# Autodesk Inventor assembly: Miras
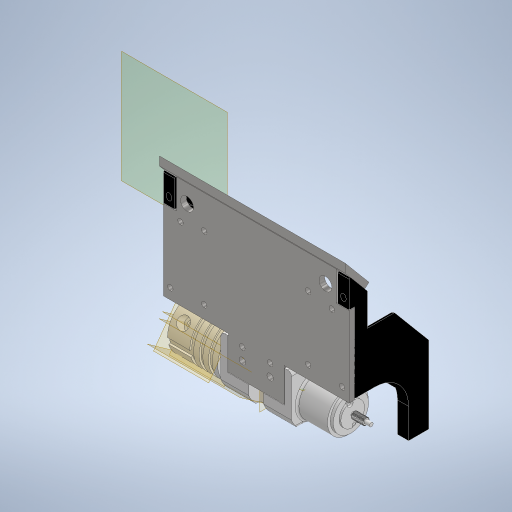
[picture p0: Inventor's stored thumbnail of the model, 512x512]
Saved by Autodesk Inventor 2023.5 (Build 275446000, 446)
## iProperties
Created: 2022-12-28
Part Number: Miras
Document SubType Name: Assembly
Designer: Kamil
Author: Kamil
## Documents named in this file (24)
- E:\PROJECTS_REPOS\Miras\mechanics\Miras.iam
- E:\PROJECTS_REPOS\Miras\mechanics\blacha_stal_3mm.ipt
- E:\PROJECTS_REPOS\Miras\mechanics\steel_2.ipt
- E:\PROJECTS_REPOS\Miras\mechanics\lead_3.ipt
- E:\PROJECTS_REPOS\Miras\mechanics\Part8.ipt
- E:\PROJECTS_REPOS\Miras\mechanics\n20 motor.ipt
- E:\PROJECTS_REPOS\Miras\mechanics\felga.ipt
- E:\PROJECTS_REPOS\Miras\mechanics\opona.ipt
- E:\PROJECTS_REPOS\Miras\mechanics\strug.ipt
- E:\PROJECTS_REPOS\Miras\mechanics\sciana.ipt
- E:\PROJECTS_REPOS\Miras\mechanics\sciana_MIR.ipt
- E:\PROJECTS_REPOS\Miras\mechanics\mirror.ipt
- E:\PROJECTS_REPOS\Miras\mechanics\uchwyt na plytke.ipt
- E:\PROJECTS_REPOS\Miras\mechanics\wachlarz_1.ipt
- E:\PROJECTS_REPOS\Miras\mechanics\montaz_wachlarzy_2.ipt
- E:\PROJECTS_REPOS\Miras\mechanics\wachlarz_1_MIR.ipt
- E:\PROJECTS_REPOS\Miras\mechanics\Serwo_z_widelcem.iam
- E:\PROJECTS_REPOS\Miras\mechanics\widelec.ipt
- E:\PROJECTS_REPOS\Miras\mechanics\faulhaber_motor.ipt
- E:\PROJECTS_REPOS\Miras\mechanics\PCB.ipt
- E:\PROJECTS_REPOS\Miras\mechanics\motors_mount_miras.ipt
- E:\PROJECTS_REPOS\Miras\mechanics\wymiar.ipt
- E:\PROJECTS_REPOS\EX_ONE_minisumo\mechanics\inventor_parts\kolo_tetsowe.ipt
- E:\PROJECTS_REPOS\Miras\mechanics\pcb_podstawka.ipt
## Components (28 placed, 23 different names)
1. blacha_stal_3mm:1 — Mate:1, Mate:2, Mate:27, Flush:4, Flush:5, Mate:28, Flush:6, Mate:30, Flush:7, Flush:22, Zestawiające:65, Kątowe:2, Równoległe:24, Równoległe:25, Równoległe:27, Równoległe:28, Zestawiające:70, Zestawiające:74, Zestawiające:75, Zestawiające:76
2. steel_2:1 — Mate:1, Mate:2, Mate:4, Mate:5, Flush:1, Zestawiające:66
3. lead_3:1 — Mate:4, Mate:5, Flush:1, Flush:2, Flush:3, Mate:16
4. Part8:1 — Flush:2, Flush:3, Mate:11, Mate:12, Mate:13, Mate:14, Mate:15, Mate:18, Mate:37, Flush:9, Flush:10, Mate:55
5. n20 motor:1 — Mate:10, Mate:11, Mate:13, Mate:14, Mate:19, Mate:20, Mate:21
6. n20 motor:2 — Mate:10, Mate:12, Mate:15, Mate:16, Mate:17, Mate:22
7. felga:1 — Mate:17, Mate:18, Mate:22, Mate:24, Mate:25
8. felga:2 — Mate:19, Mate:20, Mate:21, Mate:23, Mate:26
9. opona:1 — Mate:23, Mate:26, Zestawiające:63
10. opona:2 — Mate:24, Mate:25
11. strug:1 — Mate:27, Flush:4, Flush:5, Mate:29, Mate:31, Mate:35, Flush:21, Flush:22, Zestawiające:68, Równoległe:26
12. sciana:1 — Mate:28, Mate:29, Flush:6
13. sciana_MIR:1 — Mate:30, Flush:7, Mate:31, Flush:8, Mate:36
14. mirror:1 — Mate:35, Flush:8, Mate:36, Flush:21
15. uchwyt na plytke:1 — Mate:37, Flush:9, Flush:10, Flush:15, Mate:50, Mate:51, Mate:58
16. montaz_wachlarzy_2:1 — Flush:15, Mate:50, Mate:51, Mate:52, Mate:53, Mate:54
17. wachlarz_1:2 — Mate:52, Mate:53, Flush:16
18. wachlarz_1_MIR:1 — Mate:54, Flush:16
19. widelec:1 — Mate:55, Mate:56, Mate:57
20. Serwo_z_widelcem:1 [sub-assembly] — Mate:56, Mate:57, Mate:58
21. faulhaber_motor:1 — Kątowe:1, Zestawiające:62, Zestawiające:72
22. faulhaber_motor:2 — Kątowe:1, Zestawiające:62, Zestawiające:63, Zestawiające:71, Zestawiające:73
23. PCB:1 — Zestawiające:65, Kątowe:2, Równoległe:24, Zestawiające:66
24. motors_mount_miras:1 — Zestawiające:69, Zestawiające:70, Zestawiające:71, Zestawiające:72, Zestawiające:73
25. wymiar:1 — Zestawiające:68, Równoległe:25, Równoległe:26, Zestawiające:69
26. kolo_tetsowe:1 — Równoległe:27
27. kolo_tetsowe:2 — Równoległe:28
28. pcb_podstawka:1 — Zestawiające:74, Zestawiające:75, Zestawiające:76
## Relationships (72: Mate 51, Flush 19, Angle 2)
- Mate:1: blacha_stal_3mm:1 ↔ steel_2:1
- Mate:2: blacha_stal_3mm:1 ↔ steel_2:1
- Mate:4: steel_2:1 ↔ lead_3:1
- Mate:5: steel_2:1 ↔ lead_3:1
- Flush:1: steel_2:1 ↔ lead_3:1
- Flush:2: lead_3:1 ↔ Part8:1
- Flush:3: lead_3:1 ↔ Part8:1
- Mate:10 (5 mm): n20 motor:1 ↔ n20 motor:2
- Mate:11 (2.5 mm): Part8:1 ↔ n20 motor:1
- Mate:12: Part8:1 ↔ n20 motor:2
- Mate:13: Part8:1 ↔ n20 motor:1
- Mate:14: Part8:1 ↔ n20 motor:1
- Mate:15: Part8:1 ↔ n20 motor:2
- Mate:16: lead_3:1 ↔ n20 motor:2
- Mate:17 (0.5 mm): n20 motor:2 ↔ felga:1
- Mate:18: Part8:1 ↔ felga:1
- Mate:19 (0.5 mm): n20 motor:1 ↔ felga:2
- Mate:20: n20 motor:1 ↔ felga:2
- Mate:21: n20 motor:1 ↔ felga:2
- Mate:22: n20 motor:2 ↔ felga:1
- Mate:23: felga:2 ↔ opona:1
- Mate:24: felga:1 ↔ opona:2
- Mate:25: felga:1 ↔ opona:2
- Mate:26: felga:2 ↔ opona:1
- Mate:27: blacha_stal_3mm:1 ↔ strug:1
- Flush:4: blacha_stal_3mm:1 ↔ strug:1
- Flush:5 (2.1 mm): blacha_stal_3mm:1 ↔ strug:1
- Mate:28: blacha_stal_3mm:1 ↔ sciana:1
- Mate:29: strug:1 ↔ sciana:1
- Flush:6: blacha_stal_3mm:1 ↔ sciana:1
- Mate:30: blacha_stal_3mm:1 ↔ sciana_MIR:1
- Flush:7: blacha_stal_3mm:1 ↔ sciana_MIR:1
- Mate:31: strug:1 ↔ sciana_MIR:1
- Mate:35: strug:1 ↔ mirror:1
- Flush:8: sciana_MIR:1 ↔ mirror:1
- Mate:36: sciana_MIR:1 ↔ mirror:1
- Mate:37: Part8:1 ↔ uchwyt na plytke:1
- Flush:9: Part8:1 ↔ uchwyt na plytke:1
- Flush:10: Part8:1 ↔ uchwyt na plytke:1
- Flush:15: uchwyt na plytke:1 ↔ montaz_wachlarzy_2:1
- Mate:50: uchwyt na plytke:1 ↔ montaz_wachlarzy_2:1
- Mate:51: uchwyt na plytke:1 ↔ montaz_wachlarzy_2:1
- Mate:52: montaz_wachlarzy_2:1 ↔ wachlarz_1:2
- Mate:53: montaz_wachlarzy_2:1 ↔ wachlarz_1:2
- Mate:54: montaz_wachlarzy_2:1 ↔ wachlarz_1_MIR:1
- Flush:16: wachlarz_1:2 ↔ wachlarz_1_MIR:1
- Mate:55: Part8:1 ↔ widelec:1
- Mate:56 (0.5 mm): widelec:1 ↔ Serwo_z_widelcem:1
- Mate:57: widelec:1 ↔ Serwo_z_widelcem:1
- Mate:58: uchwyt na plytke:1 ↔ Serwo_z_widelcem:1
- Flush:21: strug:1 ↔ mirror:1
- Flush:22: blacha_stal_3mm:1 ↔ strug:1
- Kątowe:1 [Angle] (180 deg): faulhaber_motor:1 ↔ faulhaber_motor:2
- Zestawiające:62 [Mate]: faulhaber_motor:1 ↔ faulhaber_motor:2
- Zestawiające:63 [Mate]: opona:1 ↔ faulhaber_motor:2
- Zestawiające:65 [Mate] (0.5 mm): blacha_stal_3mm:1 ↔ PCB:1
- Kątowe:2 [Angle] (0 deg): blacha_stal_3mm:1 ↔ PCB:1
- Równoległe:24 [Flush] (9 mm): blacha_stal_3mm:1 ↔ PCB:1
- Zestawiające:66 [Mate]: steel_2:1 ↔ PCB:1
- Zestawiające:68 [Mate]: strug:1 ↔ wymiar:1
- Równoległe:25 [Flush]: blacha_stal_3mm:1 ↔ wymiar:1
- Równoległe:26 [Flush]: strug:1 ↔ wymiar:1
- Równoległe:27 [Flush]: blacha_stal_3mm:1 ↔ kolo_tetsowe:1
- Równoległe:28 [Flush]: blacha_stal_3mm:1 ↔ kolo_tetsowe:2
- Zestawiające:69 [Mate] (-50 mm): motors_mount_miras:1 ↔ wymiar:1
- Zestawiające:70 [Mate]: blacha_stal_3mm:1 ↔ motors_mount_miras:1
- Zestawiające:71 [Mate]: faulhaber_motor:2 ↔ motors_mount_miras:1
- Zestawiające:72 [Mate]: faulhaber_motor:1 ↔ motors_mount_miras:1
- Zestawiające:73 [Mate]: faulhaber_motor:2 ↔ motors_mount_miras:1
- Zestawiające:74 [Mate]: blacha_stal_3mm:1 ↔ pcb_podstawka:1
- Zestawiające:75 [Mate]: blacha_stal_3mm:1 ↔ pcb_podstawka:1
- Zestawiające:76 [Mate]: blacha_stal_3mm:1 ↔ pcb_podstawka:1
